# Autodesk Inventor assembly: FreundBumper
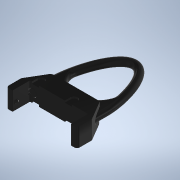
[picture p0: Inventor's stored thumbnail of the model, 180x180]
Saved by Autodesk Inventor 2020.4 (Build 244396010, 396A)
## iProperties
Created: 2021-10-09
Part Number: FreundBumper
Document SubType Name: Assembly
Designer: t-nagamine
Author: t-nagamine
## Documents named in this file (3)
- C:\Users\t-nagamine\Documents\Cit Brains\issue\IPT IAM\FreundBumper.iam
- C:\Users\t-nagamine\Documents\Cit Brains\issue\IPT IAM\FreundBumper_Stand.ipt
- C:\Users\t-nagamine\Documents\Cit Brains\issue\IPT IAM\FrontBumper_main.ipt
## Components (2 placed, 2 different names)
1. FreundBumper_Stand:1 — 挿入:1, メイト:1
2. FrontBumper_main:1 — 挿入:1, メイト:1
## Relationships (2: Insert 1, Mate 1)
- 挿入:1 [Insert]: FreundBumper_Stand:1 ↔ FrontBumper_main:1
- メイト:1 [Mate]: FreundBumper_Stand:1 ↔ FrontBumper_main:1
